# Autodesk Inventor assembly: AM14U4 Square
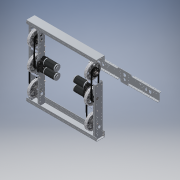
[picture p0: Inventor's stored thumbnail of the model, 180x180]
Saved by Autodesk Inventor 2017 (Build 210142000, 142)
## iProperties
Created: 2018-10-11
Part Number: AM14U4 Square
Material: 一般
Description: STEP AP214
Document SubType Name: Assembly
Designer: IJA
Sending System: SolidWorks 2018
Preprocessor: SwSTEP 2.0
Title: AM14U4 Square.STEP
Revision Number: ANY
## Documents named in this file (5)
- D:\Works\Robot2\AM14U4 Square.iam
- D:\Works\Robot2\AM14U4 Square Half.iam
- D:\Works\Robot2\am-xxxx AM14U4 Outside Plate Square_DefaultSM-FLAT-PATTERN_MIR.ipt
- D:\Works\Robot2\am-xxxx AM14U4 Outside Plate Square_DefaultSM-FLAT-PATTERN_MIR2.ipt
- D:\Works\Robot2\am-xxxx AM14U4 Inside Plate Square2.ipt
## Components (5 placed, 5 different names)
1. AM14U4 Square Half_1 [sub-assembly] — 貼合:1, 貼合:2
2. AM14U4 Square Half_2 [sub-assembly] — 角度:1, 角度:2
3. am-xxxx AM14U4 Outside Plate Square_DefaultSM-FLAT-PATTERN_MIR:1 — 貼合:1
4. am-xxxx AM14U4 Outside Plate Square_DefaultSM-FLAT-PATTERN_MIR2:1 — 角度:1, 角度:2, 貼合:2
5. am-xxxx AM14U4 Inside Plate Square2:1
## Relationships (4: Mate 2, Angle 2)
- 貼合:1 [Mate]: AM14U4 Square Half_1 ↔ am-xxxx AM14U4 Outside Plate Square_DefaultSM-FLAT-PATTERN_MIR:1
- 角度:1 [Angle] (0 deg): AM14U4 Square Half_2 ↔ am-xxxx AM14U4 Outside Plate Square_DefaultSM-FLAT-PATTERN_MIR2:1
- 角度:2 [Angle] (0 deg): AM14U4 Square Half_2 ↔ am-xxxx AM14U4 Outside Plate Square_DefaultSM-FLAT-PATTERN_MIR2:1
- 貼合:2 [Mate]: AM14U4 Square Half_1 ↔ am-xxxx AM14U4 Outside Plate Square_DefaultSM-FLAT-PATTERN_MIR2:1
